# Autodesk Inventor assembly: ENSAMBLE CUERPO PUERTA M 2020-9.5L
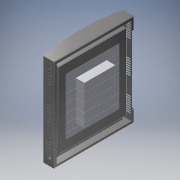
[picture p0: Inventor's stored thumbnail of the model, 180x180]
Saved by Autodesk Inventor 2017 (Build 210142000, 142)
## iProperties
Created: 2021-02-12
Part Number: ENSAMBLE CUERPO PUERTA M 2020-9.5L
Description: STEP AP203
Document SubType Name: Assembly
Designer: USUARIO
Sending System: SolidWorks 2013
Preprocessor: SwSTEP 2.0
Title: ENSAMBLE CUERPO PUERTA M 2020-9.5L.STEP
Revision Number: ANY
## Documents named in this file (9)
- D:\Laboratorio\Mufla\2021\Mufla 9L Psoc Artilab #0045884XX OP202139\Modelo\ENSAMBLE CUERPO PUERTA M 2020-9.5L.iam
- D:\Laboratorio\Mufla\2021\Mufla 9L Psoc Artilab #0045884XX OP202139\Modelo\FRONTAL PUERTA M 2020-9.5L.ipt
- D:\Laboratorio\Mufla\2021\Mufla 9L Psoc Artilab #0045884XX OP202139\Modelo\LATERAL PUERTA M 2020-9.5L.ipt
- D:\Laboratorio\Mufla\2021\Mufla 9L Psoc Artilab #0045884XX OP202139\Modelo\SOPORTE INTERIOR CONTRATAPA M 2020-9.5L.ipt
- D:\Laboratorio\Mufla\2021\Mufla 9L Psoc Artilab #0045884XX OP202139\Modelo\CONTRATAPA EXTERIOR M 2020-9.5L_PredeterminadoSM-CHAPA-DESPLEGADA.ipt
- D:\Laboratorio\Mufla\2021\Mufla 9L Psoc Artilab #0045884XX OP202139\Modelo\CONTRATAPA INTERIOR M 2020-9.5L_PredeterminadoSM-CHAPA-DESPLEGADA.ipt
- D:\Laboratorio\Mufla\2021\Mufla 9L Psoc Artilab #0045884XX OP202139\Modelo\PiezaPuerta-1.ipt
- D:\Laboratorio\Mufla\2021\Mufla 9L Psoc Artilab #0045884XX OP202139\Modelo\PiezaPuerta-2.ipt
- D:\Laboratorio\Mufla\2021\Mufla 9L Psoc Artilab #0045884XX OP202139\Modelo\PiezaPuerta-3.ipt
## Components (15 placed, 10 different names)
1. FRONTAL PUERTA M 2020-9.5L_1
2. LATERAL PUERTA M 2020-9.5L_2
3. LATERAL PUERTA M 2020-9.5L_3
4. SOPORTE INTERIOR CONTRATAPA M 2020-9.5L_4
5. SOPORTE INTERIOR CONTRATAPA M 2020-9.5L_5
6. CONTRATAPA EXTERIOR M 2020-9.5L_PredeterminadoSM-CHAPA-DESPLEGADA_6 — Mate:18
7. CONTRATAPA INTERIOR M 2020-9.5L_PredeterminadoSM-CHAPA-DESPLEGADA_7 — Mate:1, Mate:2, Mate:3, Mate:4, Mate:5, Mate:6, Mate:8, Mate:9, Mate:11, Mate:12, Mate:15, Mate:16, Mate:20, Mate:21, Mate:23, Mate:24
8. PiezaPuerta-1:1 — Mate:1, Mate:2, Mate:19
9. PiezaPuerta-2:1 — Mate:3, Mate:4, Mate:7, Mate:17
10. PiezaPuerta-2:2 — Mate:5, Mate:6, Mate:7, Mate:10
11. PiezaPuerta-2:3 — Mate:8, Mate:9, Mate:10, Mate:13
12. PiezaPuerta-2:4 — Mate:11, Mate:12, Mate:13, Mate:18, Mate:22
13. PiezaPuerta-3:1 — Mate:15, Mate:16, Mate:17, Mate:19
14. PiezaPuerta-1:2 — Mate:20, Mate:21, Mate:22, Mate:25
15. PiezaPuerta-1:3 — Mate:23, Mate:24, Mate:25
## Relationships (24: Mate 24)
- Mate:1: CONTRATAPA INTERIOR M 2020-9.5L_PredeterminadoSM-CHAPA-DESPLEGADA_7 ↔ PiezaPuerta-1:1
- Mate:2: CONTRATAPA INTERIOR M 2020-9.5L_PredeterminadoSM-CHAPA-DESPLEGADA_7 ↔ PiezaPuerta-1:1
- Mate:3: CONTRATAPA INTERIOR M 2020-9.5L_PredeterminadoSM-CHAPA-DESPLEGADA_7 ↔ PiezaPuerta-2:1
- Mate:4: CONTRATAPA INTERIOR M 2020-9.5L_PredeterminadoSM-CHAPA-DESPLEGADA_7 ↔ PiezaPuerta-2:1
- Mate:5: CONTRATAPA INTERIOR M 2020-9.5L_PredeterminadoSM-CHAPA-DESPLEGADA_7 ↔ PiezaPuerta-2:2
- Mate:6: CONTRATAPA INTERIOR M 2020-9.5L_PredeterminadoSM-CHAPA-DESPLEGADA_7 ↔ PiezaPuerta-2:2
- Mate:7 (0.5 mm): PiezaPuerta-2:1 ↔ PiezaPuerta-2:2
- Mate:8: CONTRATAPA INTERIOR M 2020-9.5L_PredeterminadoSM-CHAPA-DESPLEGADA_7 ↔ PiezaPuerta-2:3
- Mate:9: CONTRATAPA INTERIOR M 2020-9.5L_PredeterminadoSM-CHAPA-DESPLEGADA_7 ↔ PiezaPuerta-2:3
- Mate:10 (0.5 mm): PiezaPuerta-2:2 ↔ PiezaPuerta-2:3
- Mate:11: CONTRATAPA INTERIOR M 2020-9.5L_PredeterminadoSM-CHAPA-DESPLEGADA_7 ↔ PiezaPuerta-2:4
- Mate:12: CONTRATAPA INTERIOR M 2020-9.5L_PredeterminadoSM-CHAPA-DESPLEGADA_7 ↔ PiezaPuerta-2:4
- Mate:13 (0.5 mm): PiezaPuerta-2:3 ↔ PiezaPuerta-2:4
- Mate:15: CONTRATAPA INTERIOR M 2020-9.5L_PredeterminadoSM-CHAPA-DESPLEGADA_7 ↔ PiezaPuerta-3:1
- Mate:16: CONTRATAPA INTERIOR M 2020-9.5L_PredeterminadoSM-CHAPA-DESPLEGADA_7 ↔ PiezaPuerta-3:1
- Mate:17 (0.5 mm): PiezaPuerta-2:1 ↔ PiezaPuerta-3:1
- Mate:18 (105 mm): CONTRATAPA EXTERIOR M 2020-9.5L_PredeterminadoSM-CHAPA-DESPLEGADA_6 ↔ PiezaPuerta-2:4
- Mate:19 (0.5 mm): PiezaPuerta-1:1 ↔ PiezaPuerta-3:1
- Mate:20: CONTRATAPA INTERIOR M 2020-9.5L_PredeterminadoSM-CHAPA-DESPLEGADA_7 ↔ PiezaPuerta-1:2
- Mate:21: CONTRATAPA INTERIOR M 2020-9.5L_PredeterminadoSM-CHAPA-DESPLEGADA_7 ↔ PiezaPuerta-1:2
- Mate:22 (0.5 mm): PiezaPuerta-2:4 ↔ PiezaPuerta-1:2
- Mate:23: CONTRATAPA INTERIOR M 2020-9.5L_PredeterminadoSM-CHAPA-DESPLEGADA_7 ↔ PiezaPuerta-1:3
- Mate:24: CONTRATAPA INTERIOR M 2020-9.5L_PredeterminadoSM-CHAPA-DESPLEGADA_7 ↔ PiezaPuerta-1:3
- Mate:25 (0.5 mm): PiezaPuerta-1:2 ↔ PiezaPuerta-1:3
